# Autodesk Inventor assembly: wheel 2 sprocket
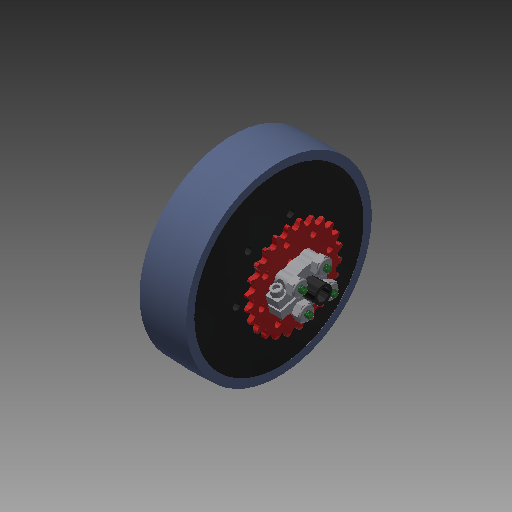
[picture p0: Inventor's stored thumbnail of the model, 512x512]
Saved by Autodesk Inventor 2018 (Build 220112000, 112)
## iProperties
Created: 2017-11-04
Part Number: wheel 2 sprocket
Document SubType Name: Assembly
Designer: ball
Author: ball
## Documents named in this file (13)
- C:\FTC\2017Robot\wheel 2 sprocket.iam
- C:\FTC\Andymark\am-2648_4inWheel8mmHub.ipt
- C:\FTC\Actobotics\545 parts\545456.ipt
- C:\FTC\Actobotics\615 parts\615106.ipt
- C:\FTC\Actobotics\545 parts\545619 assembly.ipt
- C:\FTC\Actobotics\545 parts\545619 assembly drilled out.ipt
- C:\FTC\Actobotics\545 parts\545456 counterbore.ipt
- C:\FTC\Actobotics\632 parts\632128.ipt
- C:\FTC\Actobotics\632 parts\632142.ipt
- C:\FTC\Actobotics\632 parts\632120.ipt
- C:\FTC\Actobotics\632 parts\632114.ipt
- C:\FTC\Actobotics\525 parts\625102 assembly.ipt
- C:\FTC\Actobotics\633 parts\633104.ipt
## Components (29 placed, 12 different names)
1. am-2648_4inWheel8mmHub:1 — Mate:2, Mate:3, Mate:4, Mate:11, Mate:12, Mate:13
2. 545456:1 — Mate:2, Mate:3, Mate:4, Mate:5, Mate:6, Mate:7, Mate:34, Mate:35, Mate:36, Mate:37, Mate:38, Mate:39, Mate:40, Mate:41
3. 615106:1 — Mate:5, Mate:6, Mate:7, Mate:8, Mate:9, Mate:10
4. 615106:2 — Mate:14, Mate:15, Mate:16, Mate:21, Mate:22, Mate:23
5. 545619 assembly:1 — Mate:8, Mate:9, Mate:10, Mate:45
6. 545619 assembly drilled out:1 — Mate:14, Mate:15, Mate:16, Mate:24, Mate:25, Mate:26, Mate:27, Mate:28, Mate:29, Mate:30, Mate:31, Mate:55, Mate:56
7. 545456 counterbore:1 — Mate:11, Mate:12, Mate:13, Mate:17, Mate:18, Mate:21, Mate:22, Mate:23, Mate:57, Mate:58, Mate:59, Mate:60, Mate:61, Mate:62, Mate:63, Mate:64, Mate:65, Mate:66, Mate:67, Mate:68
8. 632128:1 — Mate:17, Mate:18
9. 632120:2
10. 632142:2 — Mate:24, Mate:25
11. 632142:3 — Mate:30, Mate:31
12. 632142:4 — Mate:28, Mate:29
13. 632142:5 — Mate:26, Mate:27
14. 632114:1 — Mate:36, Mate:37
15. 632114:2 — Mate:39, Mate:41, Mate:46
16. 632114:3 — Mate:38, Mate:40
17. 632114:4 — Mate:34, Mate:35
18. 625102 assembly:3 — Mate:45, Mate:46
19. 633104:1 — Mate:47, Mate:48, Mate:49, Mate:51, Mate:53, Mate:55, Mate:56
20. 633104:2 — Mate:47, Mate:48, Mate:50
21. 633104:3 — Mate:53, Mate:54
22. 633104:4 — Mate:51, Mate:52, Mate:54
23. 633104:5 — Mate:49, Mate:50, Mate:52
24. 632120:3 — Mate:61, Mate:62
25. 632120:4 — Mate:59, Mate:60
26. 632120:5 — Mate:57, Mate:58
27. 632128:2 — Mate:63, Mate:64
28. 632128:3 — Mate:65, Mate:66
29. 632128:4 — Mate:67, Mate:68
## Relationships (62: Mate 62)
- Mate:2: am-2648_4inWheel8mmHub:1 ↔ 545456:1
- Mate:3: am-2648_4inWheel8mmHub:1 ↔ 545456:1
- Mate:4: am-2648_4inWheel8mmHub:1 ↔ 545456:1
- Mate:5: 545456:1 ↔ 615106:1
- Mate:6: 545456:1 ↔ 615106:1
- Mate:7: 545456:1 ↔ 615106:1
- Mate:8: 615106:1 ↔ 545619 assembly:1
- Mate:9: 615106:1 ↔ 545619 assembly:1
- Mate:10: 615106:1 ↔ 545619 assembly:1
- Mate:11: am-2648_4inWheel8mmHub:1 ↔ 545456 counterbore:1
- Mate:12: am-2648_4inWheel8mmHub:1 ↔ 545456 counterbore:1
- Mate:13: am-2648_4inWheel8mmHub:1 ↔ 545456 counterbore:1
- Mate:14: 615106:2 ↔ 545619 assembly drilled out:1
- Mate:15: 615106:2 ↔ 545619 assembly drilled out:1
- Mate:16: 615106:2 ↔ 545619 assembly drilled out:1
- Mate:17: 545456 counterbore:1 ↔ 632128:1
- Mate:18: 545456 counterbore:1 ↔ 632128:1
- [Mate]: 545456 counterbore:1 ↔ 632120:2
- [Mate]: 545456 counterbore:1 ↔ 632120:2
- Mate:21: 615106:2 ↔ 545456 counterbore:1
- Mate:22: 615106:2 ↔ 545456 counterbore:1
- Mate:23: 615106:2 ↔ 545456 counterbore:1
- Mate:24: 545619 assembly drilled out:1 ↔ 632142:2
- Mate:25: 545619 assembly drilled out:1 ↔ 632142:2
- Mate:26: 545619 assembly drilled out:1 ↔ 632142:5
- Mate:27: 545619 assembly drilled out:1 ↔ 632142:5
- Mate:28: 545619 assembly drilled out:1 ↔ 632142:4
- Mate:29: 545619 assembly drilled out:1 ↔ 632142:4
- Mate:30: 545619 assembly drilled out:1 ↔ 632142:3
- Mate:31: 545619 assembly drilled out:1 ↔ 632142:3
- Mate:34: 545456:1 ↔ 632114:4
- Mate:35: 545456:1 ↔ 632114:4
- Mate:36: 545456:1 ↔ 632114:1
- Mate:37: 545456:1 ↔ 632114:1
- Mate:38: 545456:1 ↔ 632114:3
- Mate:39: 545456:1 ↔ 632114:2
- Mate:40: 545456:1 ↔ 632114:3
- Mate:41: 545456:1 ↔ 632114:2
- Mate:45: 545619 assembly:1 ↔ 625102 assembly:3
- Mate:46: 632114:2 ↔ 625102 assembly:3
- Mate:47: 633104:1 ↔ 633104:2
- Mate:48: 633104:1 ↔ 633104:2
- Mate:49: 633104:1 ↔ 633104:5
- Mate:50: 633104:2 ↔ 633104:5
- Mate:51: 633104:1 ↔ 633104:4
- Mate:52: 633104:4 ↔ 633104:5
- Mate:53: 633104:1 ↔ 633104:3
- Mate:54: 633104:3 ↔ 633104:4
- Mate:55: 545619 assembly drilled out:1 ↔ 633104:1
- Mate:56: 545619 assembly drilled out:1 ↔ 633104:1
- Mate:57: 545456 counterbore:1 ↔ 632120:5
- Mate:58: 545456 counterbore:1 ↔ 632120:5
- Mate:59: 545456 counterbore:1 ↔ 632120:4
- Mate:60: 545456 counterbore:1 ↔ 632120:4
- Mate:61: 545456 counterbore:1 ↔ 632120:3
- Mate:62: 545456 counterbore:1 ↔ 632120:3
- Mate:63: 545456 counterbore:1 ↔ 632128:2
- Mate:64: 545456 counterbore:1 ↔ 632128:2
- Mate:65: 545456 counterbore:1 ↔ 632128:3
- Mate:66: 545456 counterbore:1 ↔ 632128:3
- Mate:67: 545456 counterbore:1 ↔ 632128:4
- Mate:68: 545456 counterbore:1 ↔ 632128:4
